# Autodesk Inventor assembly: 2020_ax_connector_asm
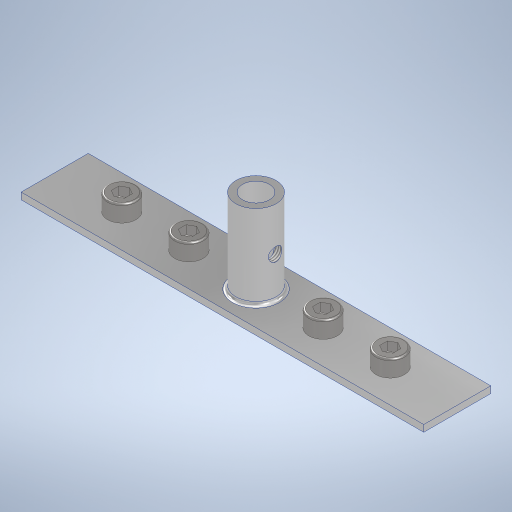
[picture p0: Inventor's stored thumbnail of the model, 512x512]
Saved by Autodesk Inventor 2024 (Build 280153000, 153)
## iProperties
Created: 2025-12-24
Part Number: 2020_ax_connector_asm
Document SubType Name: Assembly
Designer: schar
Author: schar
## Documents named in this file (4)
- C:\Users\schar\Desktop\projectBlueprint\AMSTS\hardware\2020_ax_connector_asm.iam
- C:\Users\schar\Desktop\projectBlueprint\AMSTS\hardware\2020_ax_connector.ipt
- C:\Users\schar\Desktop\projectBlueprint\AMSTS\hardware\tnut_m5_2020.ipt
- C:\Users\schar\Documents\Inventor\Content Center Files\R2024\en-US\ISO 4762(1)\DIN EN ISO 4762 - M5 x 8.ipt
## Components (9 placed, 3 different names)
1. 2020_ax_connector:1 — Rotational:1, Rotational:2, Rotational:3, Rotational:4, Mate:1, Mate:2, Mate:3, Mate:4, Mate:5, Mate:6, Mate:7, Mate:8
2. tnut_m5_2020:1 — Rotational:1
3. tnut_m5_2020:2 — Rotational:2
4. tnut_m5_2020:3 — Rotational:3
5. tnut_m5_2020:4 — Rotational:4
6. DIN EN ISO 4762 M5 x 8:1 — Mate:7, Mate:8
7. DIN EN ISO 4762 M5 x 8:2 — Mate:5, Mate:6
8. DIN EN ISO 4762 M5 x 8:3 — Mate:3, Mate:4
9. DIN EN ISO 4762 M5 x 8:4 — Mate:1, Mate:2
## Relationships (12: Mate 8, RevoluteJoint 4)
- Rotational:1 [RevoluteJoint] (0.159 mm): 2020_ax_connector:1 ↔ tnut_m5_2020:1
- Rotational:2 [RevoluteJoint] (0.159 mm): 2020_ax_connector:1 ↔ tnut_m5_2020:2
- Rotational:3 [RevoluteJoint] (0.159 mm): 2020_ax_connector:1 ↔ tnut_m5_2020:3
- Rotational:4 [RevoluteJoint] (0.159 mm): 2020_ax_connector:1 ↔ tnut_m5_2020:4
- Mate:1: 2020_ax_connector:1 ↔ DIN EN ISO 4762 M5 x 8:4
- Mate:2: 2020_ax_connector:1 ↔ DIN EN ISO 4762 M5 x 8:4
- Mate:3: 2020_ax_connector:1 ↔ DIN EN ISO 4762 M5 x 8:3
- Mate:4: 2020_ax_connector:1 ↔ DIN EN ISO 4762 M5 x 8:3
- Mate:5: 2020_ax_connector:1 ↔ DIN EN ISO 4762 M5 x 8:2
- Mate:6: 2020_ax_connector:1 ↔ DIN EN ISO 4762 M5 x 8:2
- Mate:7: 2020_ax_connector:1 ↔ DIN EN ISO 4762 M5 x 8:1
- Mate:8: 2020_ax_connector:1 ↔ DIN EN ISO 4762 M5 x 8:1
